# Autodesk Inventor assembly: Fan System
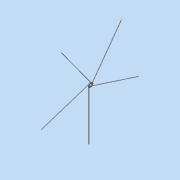
[picture p0: Inventor's stored thumbnail of the model, 180x180]
Saved by Autodesk Inventor 2015 (Build 190159000, 159)
## iProperties
Created: 2014-09-22
Part Number: Fan System
Document SubType Name: Assembly
Designer: Kris
Author: Kris
## Documents named in this file (3)
- C:\Users\Kris\Documents\Work\Inventor\drivetrain\Fan System.iam
- C:\Users\Kris\Documents\Work\Inventor\drivetrain\Bracket.ipt
- C:\Users\Kris\Documents\Work\Inventor\drivetrain\Bristle.ipt
## Components (6 placed, 2 different names)
1. Bracket:1 — Mate:1, Mate:2, Flush:1, Mate:3, Flush:2, Mate:4, Mate:5, Flush:3, Mate:6, Mate:7, Flush:4, Mate:8, Mate:9, Mate:10, Flush:5
2. Bristle:1 — Mate:1, Mate:2, Flush:1
3. Bristle:2 — Mate:7, Flush:4, Mate:8
4. Bristle:3 — Mate:5, Flush:3, Mate:6
5. Bristle:4 — Mate:9, Mate:10, Flush:5
6. Bristle:5 — Mate:3, Flush:2, Mate:4
## Relationships (15: Mate 10, Flush 5)
- Mate:1: Bracket:1 ↔ Bristle:1
- Mate:2: Bracket:1 ↔ Bristle:1
- Flush:1: Bracket:1 ↔ Bristle:1
- Mate:3: Bracket:1 ↔ Bristle:5
- Flush:2: Bracket:1 ↔ Bristle:5
- Mate:4: Bracket:1 ↔ Bristle:5
- Mate:5: Bracket:1 ↔ Bristle:3
- Flush:3: Bracket:1 ↔ Bristle:3
- Mate:6: Bracket:1 ↔ Bristle:3
- Mate:7: Bracket:1 ↔ Bristle:2
- Flush:4: Bracket:1 ↔ Bristle:2
- Mate:8: Bracket:1 ↔ Bristle:2
- Mate:9: Bracket:1 ↔ Bristle:4
- Mate:10: Bracket:1 ↔ Bristle:4
- Flush:5: Bracket:1 ↔ Bristle:4
